# Autodesk Inventor assembly: assambly onderplaat A
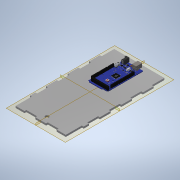
[picture p0: Inventor's stored thumbnail of the model, 180x180]
Saved by Autodesk Inventor 2021 (Build 250183000, 183)
## iProperties
Manager: Pierloot J.
Company: Emmaüs Bovenbouw Aalter
Created: 2021-01-30
Part Number: assambly onderplaat A
Catalog Web Link: http://emmausbovenbouw.op-weg.be/
Vendor: Emmaüs Bovenbouw Aalter
Document SubType Name: Assembly
Designer: Antho
Engineer: Declercq St.
Authority: Declercq St.
Title: Algemene Projecttitel
Author: Antho
## Documents named in this file (3)
- F:\GIP 6EM\Assembly\assambly onderplaat A.iam
- F:\GIP 6EM\Frame\Plaat onder.ipt
- F:\GIP 6EM\Bevestigingen\Arduino MEGA 2560 R3.ipt
## Components (2 placed, 2 different names)
1. Plaat onder:1 — Mate:1, Mate:2, Mate:3
2. Arduino MEGA 2560 R3:1 — Mate:1, Mate:2, Mate:3
## Relationships (3: Mate 3)
- Mate:1 (2 mm): Plaat onder:1 ↔ Arduino MEGA 2560 R3:1
- Mate:2: Plaat onder:1 ↔ Arduino MEGA 2560 R3:1
- Mate:3: Plaat onder:1 ↔ Arduino MEGA 2560 R3:1
